# Autodesk Inventor assembly: x_axis
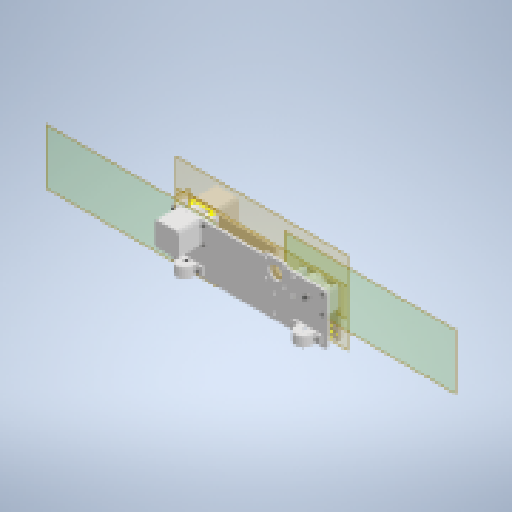
[picture p0: Inventor's stored thumbnail of the model, 512x512]
Saved by Autodesk Inventor 2024 (Build 280153000, 153)
## iProperties
Created: 2026-02-04
Part Number: x_axis
Document SubType Name: Assembly
Designer: SEMEN
Author: SEMEN
## Documents named in this file (16)
- C:\Users\SEMEN\Documents\ETZ2.0\construction\x_axis.iam
- C:\Users\SEMEN\Documents\ETZ2.0\construction\motor_x.ipt
- C:\Users\SEMEN\Documents\ETZ2.0\construction\plate_1.ipt
- C:\Users\SEMEN\Documents\ETZ2.0\construction\x_axis\Design Accelerator\Spur Gears1.iam
- C:\Users\SEMEN\Documents\ETZ2.0\construction\x_axis\Design Accelerator\Spur Gears2.iam
- C:\Users\SEMEN\Documents\Inventor\Content Center Files\R2024\en-US\GOST 8338-75\Bearing 23 GOST 8338-75.ipt
- C:\Users\SEMEN\Documents\ETZ2.0\construction\plate_2.ipt
- C:\Users\SEMEN\Documents\Inventor\Content Center Files\R2024\en-US\ISO 7045  H\ISO 7045 - M5 x 35_ - 4.8 - H - ISO.ipt
- C:\Users\SEMEN\Documents\Inventor\Content Center Files\R2024\en-US\ISO 4032(2)\ISO 4032 - M5 - ISO.ipt
- C:\Users\SEMEN\Documents\ETZ2.0\construction\plate_washer_1.ipt
- C:\Users\SEMEN\Documents\Inventor\Content Center Files\R2024\en-US\ISO 7046-1 H(1)\ISO 7046-1 - M3 x 30_ - 4.8 - H - ISO.ipt
- C:\Users\SEMEN\Documents\Inventor\Content Center Files\R2024\en-US\ISO 4032(2)\ISO 4032 - M3 - ISO.ipt
- C:\Users\SEMEN\Documents\ETZ2.0\construction\profile_bearing.ipt
- C:\Users\SEMEN\Documents\ETZ2.0\construction\bearing_holder.ipt
- C:\Users\SEMEN\Documents\Inventor\Content Center Files\R2024\en-US\ISO 7046-1 H(1)\ISO 7046-1 - M3 x 12_ - 4.8 - H - ISO.ipt
- C:\Users\SEMEN\Documents\ETZ2.0\construction\tumbler_holdeerr.ipt
## Components (49 placed, 14 different names)
1. motor_x:1 — Flush:1, Flush:2, Mate:1
2. plate_1:1 — Flush:1, Flush:2, Mate:2, Mate:3, Mate:4, Mate:9, Mate:10, Mate:11, Mate:30, Tangent:1, Flush:10, Mate:31, Tangent:2, Mate:32, Mate:33, Mate:34, Mate:42, Mate:43, Mate:44, Mate:45, Mate:46, Mate:48, Mate:50, Mate:52, Mate:67, Mate:68, Mate:69, Mate:70, Mate:71, Mate:72, Mate:75, Mate:76, Mate:77, Mate:78, Mate:79, Mate:80, Mate:85, Mate:87, Mate:89, Mate:91, Mate:93, Mate:95, Mate:107
3. Spur Gears:1 [sub-assembly] — Mate:1, Mate:4
4. Spur Gears:2 [sub-assembly] — Mate:2, Mate:3, Mate:13, Mate:15, Flush:6, Flush:7
5. plate_2:1 — Flush:5, Mate:12, Mate:35, Mate:36, Mate:37, Mate:38, Tangent:3, Mate:39, Mate:40, Mate:41, Mate:54, Mate:55, Mate:56, Mate:57, Mate:58, Mate:60, Mate:62, Mate:64, Mate:86, Mate:88, Mate:90, Mate:92, Mate:94, Mate:96, Mate:103, Mate:104, Mate:105, Flush:11, Flush:12
6. ISO 7045 H M5 x 35 - 4.8 - H:1 — Mate:9, Mate:10
7. ISO 4032 M5:1 — Mate:11, Mate:12
8. Bearing GOST 8338-75 23:1 — Mate:13, Flush:6
9. Bearing GOST 8338-75 23:2 — Mate:15, Flush:7
10. profile_bearing:1 — Mate:30, Tangent:1
11. bearing_holder:1 — Flush:10
12. profile_bearing:2 — Mate:31, Tangent:2
13. bearing_holder:2 — Mate:32, Mate:33, Mate:34, Mate:47, Mate:49, Mate:51, Mate:53
14. profile_bearing:3 — Mate:38, Tangent:3
15. bearing_holder:3 — Mate:35, Mate:36, Mate:37, Mate:59, Mate:61, Mate:63, Mate:65
16. bearing_holder:4 — Mate:39, Mate:40, Mate:41
17. ISO 7046-1 H M3 x 12 - 4.8 - H:1 — Mate:42
18. ISO 4032 M3:5 — Mate:46, Mate:47
19. ISO 7046-1 H M3 x 12 - 4.8 - H:2 — Mate:43
20. ISO 7046-1 H M3 x 12 - 4.8 - H:3 — Mate:44
21. ISO 7046-1 H M3 x 12 - 4.8 - H:4 — Mate:45
22. ISO 4032 M3:6 — Mate:48, Mate:49
23. ISO 4032 M3:7 — Mate:50, Mate:51
24. ISO 4032 M3:8 — Mate:52, Mate:53
25. ISO 7046-1 H M3 x 12 - 4.8 - H:5 — Mate:54
26. ISO 4032 M3:9 — Mate:58, Mate:59
27. ISO 7046-1 H M3 x 12 - 4.8 - H:6 — Mate:55
28. ISO 7046-1 H M3 x 12 - 4.8 - H:7 — Mate:56
29. ISO 7046-1 H M3 x 12 - 4.8 - H:8 — Mate:57
30. ISO 4032 M3:10 — Mate:60, Mate:61
31. ISO 4032 M3:11 — Mate:62, Mate:63
32. ISO 4032 M3:12 — Mate:64, Mate:65
33. plate_washer_1:3 — Mate:67, Mate:68, Mate:69
34. plate_washer_1:4 — Mate:70, Mate:71, Mate:72
35. ISO 7046-1 H M3 x 30 - 4.8 - H:3 — Mate:75
36. ISO 7046-1 H M3 x 30 - 4.8 - H:4 — Mate:76
37. ISO 7046-1 H M3 x 30 - 4.8 - H:5 — Mate:77, Mate:108
38. ISO 7046-1 H M3 x 30 - 4.8 - H:6 — Mate:78, Mate:106
39. ISO 7046-1 H M3 x 30 - 4.8 - H:7 — Mate:79
40. ISO 7046-1 H M3 x 30 - 4.8 - H:8 — Mate:80
41. ISO 4032 M3:15 — Mate:85, Mate:86
42. ISO 4032 M3:16 — Mate:87, Mate:88
43. ISO 4032 M3:17 — Mate:89, Mate:90
44. ISO 4032 M3:18 — Mate:91, Mate:92
45. ISO 4032 M3:19 — Mate:93, Mate:94
46. ISO 4032 M3:20 — Mate:95, Mate:96
47. motor_x:2 — Mate:103, Mate:104, Mate:105
48. plate_washer_1:5 — Mate:106, Mate:107, Mate:108
49. tumbler_holdeerr:1 — Flush:11, Flush:12
## Relationships (87: Mate 76, Flush 8, Tangent 3)
- Flush:1: motor_x:1 ↔ plate_1:1
- Flush:2: motor_x:1 ↔ plate_1:1
- Mate:1: motor_x:1 ↔ Spur Gears:1
- Mate:2: plate_1:1 ↔ Spur Gears:2
- Mate:3 (1 mm): plate_1:1 ↔ Spur Gears:2
- Mate:4 (1 mm): plate_1:1 ↔ Spur Gears:1
- Flush:5 (22 mm): plate_2:1
- Mate:9: plate_1:1 ↔ ISO 7045 H M5 x 35 - 4.8 - H:1
- Mate:10: plate_1:1 ↔ ISO 7045 H M5 x 35 - 4.8 - H:1
- Mate:11: plate_1:1 ↔ ISO 4032 M5:1
- Mate:12: plate_2:1 ↔ ISO 4032 M5:1
- Mate:13: Spur Gears:2 ↔ Bearing GOST 8338-75 23:1
- Mate:15: Spur Gears:2 ↔ Bearing GOST 8338-75 23:2
- Flush:6: Spur Gears:2 ↔ Bearing GOST 8338-75 23:1
- Flush:7: Spur Gears:2 ↔ Bearing GOST 8338-75 23:2
- Mate:30 (0.5 mm): plate_1:1 ↔ profile_bearing:1
- Tangent:1: plate_1:1 ↔ profile_bearing:1
- Flush:10: plate_1:1 ↔ bearing_holder:1
- Mate:31 (0.5 mm): plate_1:1 ↔ profile_bearing:2
- Tangent:2: plate_1:1 ↔ profile_bearing:2
- Mate:32: plate_1:1 ↔ bearing_holder:2
- Mate:33: plate_1:1 ↔ bearing_holder:2
- Mate:34: plate_1:1 ↔ bearing_holder:2
- Mate:35: plate_2:1 ↔ bearing_holder:3
- Mate:36: plate_2:1 ↔ bearing_holder:3
- Mate:37: plate_2:1 ↔ bearing_holder:3
- Mate:38 (0.5 mm): plate_2:1 ↔ profile_bearing:3
- Tangent:3: plate_2:1 ↔ profile_bearing:3
- Mate:39: plate_2:1 ↔ bearing_holder:4
- Mate:40: plate_2:1 ↔ bearing_holder:4
- Mate:41: plate_2:1 ↔ bearing_holder:4
- Mate:42: plate_1:1 ↔ ISO 7046-1 H M3 x 12 - 4.8 - H:1
- Mate:43: plate_1:1 ↔ ISO 7046-1 H M3 x 12 - 4.8 - H:2
- Mate:44: plate_1:1 ↔ ISO 7046-1 H M3 x 12 - 4.8 - H:3
- Mate:45: plate_1:1 ↔ ISO 7046-1 H M3 x 12 - 4.8 - H:4
- Mate:46: plate_1:1 ↔ ISO 4032 M3:5
- Mate:47: bearing_holder:2 ↔ ISO 4032 M3:5
- Mate:48: plate_1:1 ↔ ISO 4032 M3:6
- Mate:49: bearing_holder:2 ↔ ISO 4032 M3:6
- Mate:50: plate_1:1 ↔ ISO 4032 M3:7
- Mate:51: bearing_holder:2 ↔ ISO 4032 M3:7
- Mate:52: plate_1:1 ↔ ISO 4032 M3:8
- Mate:53: bearing_holder:2 ↔ ISO 4032 M3:8
- Mate:54: plate_2:1 ↔ ISO 7046-1 H M3 x 12 - 4.8 - H:5
- Mate:55: plate_2:1 ↔ ISO 7046-1 H M3 x 12 - 4.8 - H:6
- Mate:56: plate_2:1 ↔ ISO 7046-1 H M3 x 12 - 4.8 - H:7
- Mate:57: plate_2:1 ↔ ISO 7046-1 H M3 x 12 - 4.8 - H:8
- Mate:58: plate_2:1 ↔ ISO 4032 M3:9
- Mate:59: bearing_holder:3 ↔ ISO 4032 M3:9
- Mate:60: plate_2:1 ↔ ISO 4032 M3:10
- Mate:61: bearing_holder:3 ↔ ISO 4032 M3:10
- Mate:62: plate_2:1 ↔ ISO 4032 M3:11
- Mate:63: bearing_holder:3 ↔ ISO 4032 M3:11
- Mate:64: plate_2:1 ↔ ISO 4032 M3:12
- Mate:65: bearing_holder:3 ↔ ISO 4032 M3:12
- Mate:67: plate_1:1 ↔ plate_washer_1:3
- Mate:68: plate_1:1 ↔ plate_washer_1:3
- Mate:69: plate_1:1 ↔ plate_washer_1:3
- Mate:70: plate_1:1 ↔ plate_washer_1:4
- Mate:71: plate_1:1 ↔ plate_washer_1:4
- Mate:72: plate_1:1 ↔ plate_washer_1:4
- Mate:75: plate_1:1 ↔ ISO 7046-1 H M3 x 30 - 4.8 - H:3
- Mate:76: plate_1:1 ↔ ISO 7046-1 H M3 x 30 - 4.8 - H:4
- Mate:77: plate_1:1 ↔ ISO 7046-1 H M3 x 30 - 4.8 - H:5
- Mate:78: plate_1:1 ↔ ISO 7046-1 H M3 x 30 - 4.8 - H:6
- Mate:79: plate_1:1 ↔ ISO 7046-1 H M3 x 30 - 4.8 - H:7
- Mate:80: plate_1:1 ↔ ISO 7046-1 H M3 x 30 - 4.8 - H:8
- Mate:85: plate_1:1 ↔ ISO 4032 M3:15
- Mate:86: plate_2:1 ↔ ISO 4032 M3:15
- Mate:87: plate_1:1 ↔ ISO 4032 M3:16
- Mate:88: plate_2:1 ↔ ISO 4032 M3:16
- Mate:89: plate_1:1 ↔ ISO 4032 M3:17
- Mate:90: plate_2:1 ↔ ISO 4032 M3:17
- Mate:91: plate_1:1 ↔ ISO 4032 M3:18
- Mate:92: plate_2:1 ↔ ISO 4032 M3:18
- Mate:93: plate_1:1 ↔ ISO 4032 M3:19
- Mate:94: plate_2:1 ↔ ISO 4032 M3:19
- Mate:95: plate_1:1 ↔ ISO 4032 M3:20
- Mate:96: plate_2:1 ↔ ISO 4032 M3:20
- Mate:103: plate_2:1 ↔ motor_x:2
- Mate:104: plate_2:1 ↔ motor_x:2
- Mate:105: plate_2:1 ↔ motor_x:2
- Mate:106: ISO 7046-1 H M3 x 30 - 4.8 - H:6 ↔ plate_washer_1:5
- Mate:107: plate_1:1 ↔ plate_washer_1:5
- Mate:108: ISO 7046-1 H M3 x 30 - 4.8 - H:5 ↔ plate_washer_1:5
- Flush:11: plate_2:1 ↔ tumbler_holdeerr:1
- Flush:12: plate_2:1 ↔ tumbler_holdeerr:1
